# Autodesk Inventor assembly: CPLSC20-8-8
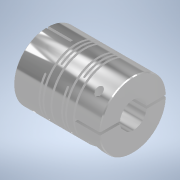
[picture p0: Inventor's stored thumbnail of the model, 180x180]
Saved by Autodesk Inventor 2022.3 (Build 263350000, 350)
## iProperties
Category: PARTsolutions
Company: MISUMI
Part Number: CPLSC20-8-8
Catalog Web Link: www.cadenas.de
Description: CPLCN, CPLSC-Couplings - Slit, Clamping - Normal
Vendor: MISUMI
Document SubType Name: Assembly
Designer: partserver
Manufacturer: MISUMI
Mass: 5.52302 g
Surface Area: 66.8281 cm^2
Volume: 5.52302 cm^3
Density: 1 g/cm^3
PSOL_IDENT_0: {$CADENAS_DATA\23d-libs\misumi\metric\50_couplings\cplcn_asmtab.prj},209 {VTYP=3D},{STYP=ASSTAB},{NB=
PSOL_IDENT_1: CPLSC20-8-8},{LINA=CPLSC20-8-8},{NN=CPLCN, CPLSC},{DATE=09.09.2019 15:28:28},{GEOMDATE=09.12.2013},{
PSOL_IDENT_2: VERSION=},{LINEID=20},{WBVAR=MAT,ALT1,LDC,DD1,ALT2,RDC,DD2},{WBNUMERIC=LDC,RDC}  {NB=CPLSC20-8-8},{L
PSOL_IDENT_3: INA=CPLSC20-8-8},{KT=DUMMY},{PN=CPLSC20-8-8},{MAT=1},{ST=-},{AC=Hex Socket Head Cap Screw},{TYPE=CPL
PSOL_IDENT_4: SC},{D=20},{DDIA=20.000},{D1='5','5','6','6','6.35','6.35','8','8'},{ALT1=},{ALT1ALG=},{ALT1ALG2= ''
PSOL_IDENT_5: , 'w/o LDC (Shaft Hole Diameter Left Shaft)', 'LDC','with LDC (Shaft Hole Diameter Left Shaft)' },{D
PSOL_IDENT_6: LALT1=8},{LDC=0.000},{LDCALG=0},{LDCALG1=0.0},{LDCMIN=5},{DD1=8},{DD11=8},{DD1ALG1='5','5','6','6','
PSOL_IDENT_7: 6.35','6.35','8','8'},{DD1ALG2=8},{D2='8','8'},{ALT2=},{ALT2ALG=},{ALT2ALG1= '', 'w/o RDC (Shaft Hol
PSOL_IDENT_8: e Diameter Right Shaft)', 'RDC'  , 'with RDC (Shaft Hole Diameter Right Shaft)' },{RDC=0.000},{RDCAL
PSOL_IDENT_9: G=[0]},{RDCALG1=0.0},{DD2=8},{DD2ALG1='8','8'},{DD2ALG11='6','6','6.35','6.35','8','8'},{DD2ALG2=8},
PSOL_IDENT_10: {DL=8},{DR=8},{DD3=8.5},{L=26},{L1=26.000},{LL=7.5},{LL1=7.500},{M=2.5},{TSIMD=2.500},{TSIMIN=2.013}
PSOL_IDENT_11: ,{A=6.5},{A1=6.500},{F=3.75},{F1=3.750},{TSI=M2.5},{SC1=2.0000},{SC2=8.0000},{L2=6.800},{L3=0.600},{
PSOL_IDENT_12: L4=15.600},{L5=0.800},{L6=1.200},{TSI1=4.900},{ALTALG2='','Select RDC'},{PPATH=cplcn_temp.prj},{NO=1
PSOL_IDENT_13: .000}
NB: CPLSC20-8-8
NN: CPLCN, CPLSC
NT: Couplings - Slit, Clamping - Normal
NBSYN: $PN.
LINA: CPLSC20-8-8
CATALOG: Misumi
PN: CPLSC20-8-8
MAT: Stainless Steel
ST: -
AC: Hex Socket Head Cap Screw
D: 20
ALT1: w/o LDC (Shaft Hole Diameter Left Shaft)
LDC: 0
DD1: 8
ALT2: w/o RDC (Shaft Hole Diameter Right Shaft)
RDC: 0
DD2: 8
L: 26
LL: 7.5
M: 2.5
A: 6.5
F: 3.75
SUPPLIER: MISUMI
ARTICLENO: CPLSC20-8-8
BOMINFO: CPLSC20-8-8
CREATOR: CADENAS GmbH
Title: CPLSC20-8-8
Author: Cadenas PARTsolutions
Comments: Couplings - Slit, Clamping - Normal
## Documents named in this file (3)
- C:\Users\YusukeKunita\Documents\GrabCAD\Development\BasicParts\Coupling\CPLSC20-8-8\CPLSC20-8-8.iam
- C:\Users\YusukeKunita\Documents\GrabCAD\Development\BasicParts\Coupling\CPLSC20-8-8\CPLSC20-8-8_b.ipt
- C:\Users\YusukeKunita\Documents\GrabCAD\Development\BasicParts\Coupling\CPLSC20-8-8\M2_5.ipt
## Components (3 placed, 2 different names)
1. CPLSC20-8-8_b:1 — L2_XY@1 <-> SCW_XY@2, L2_Z@1 <-> SCW_Z@2, L2_YZ@1 <-> SCW_YZ@2, R2_XY@1 <-> SCW_XY@3, R2_Z@1 <-> SCW_Z@3, R2_YZ@1 <-> SCW_YZ@3
2. M2_5:1 — L2_XY@1 <-> SCW_XY@2, L2_Z@1 <-> SCW_Z@2, L2_YZ@1 <-> SCW_YZ@2
3. M2_5:2 — R2_XY@1 <-> SCW_XY@3, R2_Z@1 <-> SCW_Z@3, R2_YZ@1 <-> SCW_YZ@3
## Relationships (6: Mate 4, Angle 2)
- L2_XY@1 <-> SCW_XY@2 [Mate]: CPLSC20-8-8_b:1 ↔ M2_5:1
- L2_Z@1 <-> SCW_Z@2 [Mate]: CPLSC20-8-8_b:1 ↔ M2_5:1
- L2_YZ@1 <-> SCW_YZ@2 [Angle] (0 deg): CPLSC20-8-8_b:1 ↔ M2_5:1
- R2_XY@1 <-> SCW_XY@3 [Mate]: CPLSC20-8-8_b:1 ↔ M2_5:2
- R2_Z@1 <-> SCW_Z@3 [Mate]: CPLSC20-8-8_b:1 ↔ M2_5:2
- R2_YZ@1 <-> SCW_YZ@3 [Angle] (0 deg): CPLSC20-8-8_b:1 ↔ M2_5:2
